# Autodesk Inventor assembly: CL-6HX-A
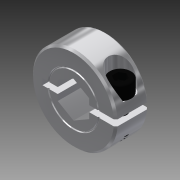
[picture p0: Inventor's stored thumbnail of the model, 180x180]
Saved by Autodesk Inventor 2016 SP1 (Build 200210100, 210)
## iProperties
Category: Miscellaneous
Company: Autodesk Inc.
Created: 2015-12-04
Part Number: CL-6HX-A
Document SubType Name: Assembly
Designer: Autodesk Inc.
Catalog Web Link: http://www.ruland.com/shaft-collar.php?recordID=CL-6HX-A
Vendor: Ruland Manufacturing
Author: Autodesk Inc.
## Documents named in this file (3)
- D:\FIRST\FRC KOP 2016\FRC KOP 2016\Miscellaneous\MISC_ShaftCollar_CL-6HX-A.iam
- D:\FIRST\FRC KOP 2016\FRC KOP 2016\Miscellaneous\Parts\MISC_ShaftCollar_CL-6HX-A.ipt
- D:\FIRST\FRC KOP 2016\FRC KOP 2016\Miscellaneous\Parts\ANSI B18.3 - 6-32 UNC - 0.375(31).ipt
## Components (2 placed, 2 different names)
1. MISC_ShaftCollar_CL-6HX-A:1 — Insert:1
2. Hexagon Socket Head Cap Screw - Inch No. 6 - 32 UNC - 3/8:1 — Insert:1
## Relationships (1: Insert 1)
- Insert:1: MISC_ShaftCollar_CL-6HX-A:1 ↔ Hexagon Socket Head Cap Screw - Inch No. 6 - 32 UNC - 3/8:1
